# Autodesk Inventor assembly: Zespół1
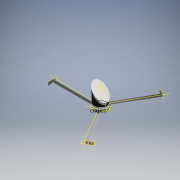
[picture p0: Inventor's stored thumbnail of the model, 180x180]
Saved by Autodesk Inventor 2019.4 (Build 234330000, 330)
## iProperties
Created: 2019-05-27
Part Number: Zespół1
Material: Ogólny
Document SubType Name: Assembly
Designer: barto
Author: barto
## Documents named in this file (9)
- F:\GOTOWY BEM\SECONDARYMIRROR2\Zespół1.iam
- F:\GOTOWY BEM\SECONDARYMIRROR2\Część1.ipt
- F:\GOTOWY BEM\SECONDARYMIRROR2\podporka_pajaka.ipt
- F:\GOTOWY BEM\SECONDARYMIRROR2\trzymadlo.ipt
- F:\GOTOWY BEM\SECONDARYMIRROR2\srodek_pajaka.ipt
- F:\GOTOWY BEM\SECONDARYMIRROR2\wkret_z_kulka.ipt
- F:\GOTOWY BEM\SECONDARYMIRROR2\ramie_pajaka.ipt
- F:\GOTOWY BEM\SECONDARYMIRROR2\Bolted Connection1.iam
- F:\GOTOWY BEM\SECONDARYMIRROR2\Bolted Connection3.iam
## Components (14 placed, 7 different names)
1. Część1:1 — Zestawiający:1, Zestawiający:2
2. podporka_pajaka:1 — Zestawiający:4, Zestawiający:5, 0,95, Mate:16, Mate:17, Mate:18, Mate:24
3. trzymadlo:1 — Zestawiający:1, Zestawiający:2, Zestawiający:4, Zestawiający:5, Mate:24
4. srodek_pajaka:1 — Zestawiający:9, Równoległy:1, Styczny:1, Mate:16, Mate:17, Mate:18, Mate:19, Mate:20, Tangent:2, Mate:25
5. wkret_z_kulka:1 — Zestawiający:9, 0,95
6. ramie_pajaka:1 — Równoległy:1, Styczny:1, Mate:21, Mate:25
7. ramie_pajaka:2 — Mate:26, Mate:27
8. ramie_pajaka:3
9. Bolted Connection:1 [sub-assembly] — Mate:19, Mate:20
10. Bolted Connection:2 [sub-assembly]
11. Bolted Connection:3 [sub-assembly]
12. Bolted Connection:4 [sub-assembly] — Mate:26, Mate:27
13. Bolted Connection:5 [sub-assembly]
14. Bolted Connection:6 [sub-assembly]
## Component patterns: (3 elements, first: ramie_pajaka:1), (3 elements, first: Bolted Connection:1), (3 elements, first: Bolted Connection:4)
## Relationships (19: Mate 16, Tangent 2, Flush 1)
- Zestawiający:1 [Mate]: Część1:1 ↔ trzymadlo:1
- Zestawiający:2 [Mate]: Część1:1 ↔ trzymadlo:1
- Zestawiający:4 [Mate]: podporka_pajaka:1 ↔ trzymadlo:1
- Zestawiający:5 [Mate]: podporka_pajaka:1 ↔ trzymadlo:1
- Zestawiający:9 [Mate]: srodek_pajaka:1 ↔ wkret_z_kulka:1
- 0,95 [Mate] (0.981 mm): podporka_pajaka:1 ↔ wkret_z_kulka:1
- Równoległy:1 [Flush]: srodek_pajaka:1 ↔ ramie_pajaka:1
- Styczny:1 [Tangent]: srodek_pajaka:1 ↔ ramie_pajaka:1
- Mate:16 (2 mm): podporka_pajaka:1 ↔ srodek_pajaka:1
- Mate:17: podporka_pajaka:1 ↔ srodek_pajaka:1
- Mate:18: podporka_pajaka:1 ↔ srodek_pajaka:1
- Mate:19: srodek_pajaka:1 ↔ Bolted Connection:1
- Mate:20: srodek_pajaka:1 ↔ Bolted Connection:1
- Mate:21: ramie_pajaka:1
- Tangent:2: srodek_pajaka:1
- Mate:24: podporka_pajaka:1 ↔ trzymadlo:1
- Mate:25: srodek_pajaka:1 ↔ ramie_pajaka:1
- Mate:26: ramie_pajaka:2 ↔ Bolted Connection:4
- Mate:27: ramie_pajaka:2 ↔ Bolted Connection:4
